# Autodesk Inventor assembly: __VK_Hub-Station
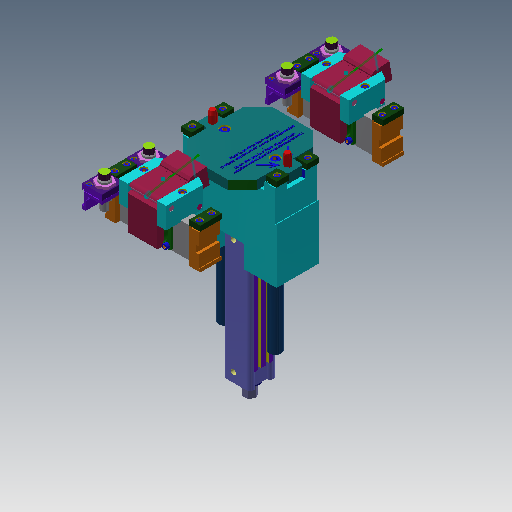
[picture p0: Inventor's stored thumbnail of the model, 512x512]
Saved by Autodesk Inventor 2019 (Build 230136000, 136)
## iProperties
Created: 2023-11-18
Part Number: __VK_Hub-Station
Material: Generisch
Document SubType Name: Assembly
Designer: RP
Author: RP
## Documents named in this file (3)
- C:\Users\RP\Documents\Inventor\Projekt_Angelspule\_Verkettung\_VK_Hub-Station.iam
- C:\Users\RP\Documents\Inventor\Projekt_Angelspule\_Verkettung\__VK_Hubeinehit_100.iam
- C:\Users\RP\Documents\Inventor\Projekt_Angelspule\_Verkettung\__VK_Stopper_Vor-Stopper_Einheit_erweitert.iam
## Components (2 placed, 2 different names)
1. __VK_Stopper_Vor-Stopper_Einheit_erweitert:1 [sub-assembly]
2. __VK_Hubeinehit_100:1 [sub-assembly] — Fluchtend:1, Fluchtend:6, Fluchtend:12
## Relationships (3: Flush 3)
- Fluchtend:1 [Flush]: __VK_Hubeinehit_100:1
- Fluchtend:6 [Flush]: __VK_Hubeinehit_100:1
- Fluchtend:12 [Flush]: __VK_Hubeinehit_100:1
